# Autodesk Inventor assembly: GT2 40T 8 Bore
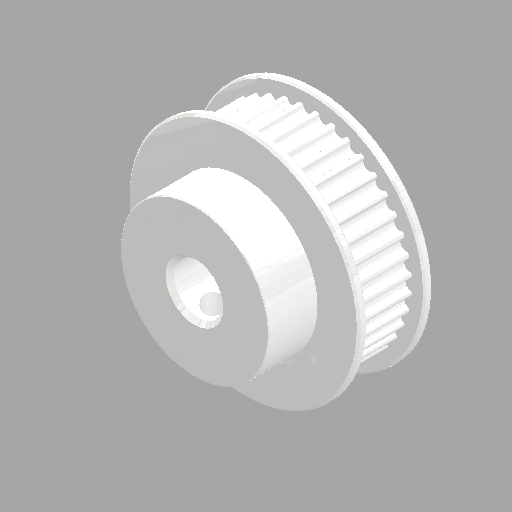
[picture p0: Inventor's stored thumbnail of the model, 512x512]
Saved by Autodesk Inventor 2025 (Build 290162000, 162)
## iProperties
Created: 2020-08-06
Part Number: GT2 40T 8 Bore
Document SubType Name: Assembly
Designer: Artem Sannikov
Title: C:/Users/Alfredo/Desktop/GT2 40T 8 Bore v2.step
Sending System: Autodesk Translation Framework v9.3.0.1241
Preprocessor: ST-DEVELOPER v18.1
## Documents named in this file (3)
- C:\Users\Artem Sannikov\Desktop\Two_axis_gimbal\3D_модели\Основная сборка\GT2 40T 8 Bore v2.iam
- C:\Users\Artem Sannikov\Desktop\Two_axis_gimbal\3D_модели\Основная сборка\Pulley.ipt
- C:\Users\Artem Sannikov\Desktop\Two_axis_gimbal\3D_модели\Основная сборка\Screw v1.ipt
## Components (2 placed, 2 different names)
1. Pulley:1 — Совмещение:1
2. Screw v1:1 — Совмещение:1
## Relationships (1: Mate 1)
- Совмещение:1 [Mate]: Pulley:1 ↔ Screw v1:1
